# Autodesk Inventor assembly: Opentrons_Microscope_v0
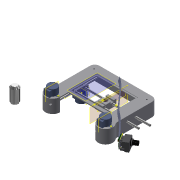
[picture p0: Inventor's stored thumbnail of the model, 180x180]
Saved by Autodesk Inventor 2019.4 (Build 234330000, 330)
## iProperties
Created: 2020-10-06
Part Number: Opentrons_Microscope_v0
Document SubType Name: Assembly
Designer: diederichbenedict
Author: diederichbenedict
## Documents named in this file (15)
- C:\Users\diederichbenedict\Dropbox\Dokumente\Promotion\PROJECTS\OPENTRONS\INVENTOR\Opentrons_Microscope_v0.iam
- C:\Users\diederichbenedict\Dropbox\Dokumente\Promotion\PROJECTS\STORMoChip\GITHUB\CAD\Nanoscopy-on-the-cheap\Workspace\00_Opticsmodule_openflexure.ipt
- C:\Users\diederichbenedict\Dropbox\Dokumente\Promotion\PROJECTS\OPENTRONS\INVENTOR\00_MTP_96-welplate.ipt
- C:\Users\diederichbenedict\Dropbox\Dokumente\Promotion\PROJECTS\OPENTRONS\INVENTOR\00_IGUS_Drylin_RJ4JP-01-06.ipt
- C:\Users\diederichbenedict\Dropbox\Dokumente\Promotion\PROJECTS\OPENTRONS\INVENTOR\00_Stepper_Motor_28BYJ-48.ipt
- C:\Users\diederichbenedict\Dropbox\Dokumente\Promotion\PROJECTS\OPENTRONS\INVENTOR\00_Thorlabs_Rod_150mm.ipt
- C:\Users\diederichbenedict\Dropbox\Dokumente\Promotion\PROJECTS\STORMoChip\GITHUB\CAD\Nanoscopy-on-the-cheap\Workspace\00_BD-DRIVE_PULLEY.ipt
- C:\Users\diederichbenedict\Dropbox\Dokumente\Promotion\PROJECTS\STORMoChip\GITHUB\CAD\Nanoscopy-on-the-cheap\Workspace\00_BD-IDLE_PULLEY.ipt
- C:\Users\diederichbenedict\Dropbox\Dokumente\Promotion\PROJECTS\OPENTRONS\INVENTOR\00_Microscope_Objective_Lens10x.ipt
- C:\Users\diederichbenedict\Dropbox\Dokumente\Promotion\PROJECTS\OPENTRONS\INVENTOR\00_Thorlabs_Rod_200mm.ipt
- C:\Users\diederichbenedict\Dropbox\Dokumente\Promotion\PROJECTS\OPENTRONS\INVENTOR\01_OTmic_BASE_v0.ipt
- C:\Users\diederichbenedict\Dropbox\Dokumente\Promotion\PROJECTS\OPENTRONS\INVENTOR\02_OTmicro_slide_y.ipt
- C:\Users\diederichbenedict\Dropbox\Dokumente\Promotion\PROJECTS\OPENTRONS\INVENTOR\03_OTmic_belt_gear.ipt
- C:\Users\diederichbenedict\Dropbox\Dokumente\Promotion\PROJECTS\OPENTRONS\INVENTOR\04_OT_mic_slide_x.ipt
- C:\Users\diederichbenedict\Dropbox\Dokumente\Promotion\PROJECTS\OPENTRONS\INVENTOR\Assembly_Opentrons_opticsmodule.iam
## Components (25 placed, 14 different names)
1. 00_Opticsmodule_openflexure:1
2. 00_MTP_96-welplate:1 — Flush:1, Flush:7, Flush:8
3. 00_Stepper_Motor_28BYJ-48:1 — Insert:2, Mate:5
4. 00_Stepper_Motor_28BYJ-48:2 — Insert:4, Mate:7
5. 00_Thorlabs_Rod_150mm:3 — Insert:1, Mate:6, Mate:9
6. 00_Thorlabs_Rod_150mm:4 — Insert:3, Mate:8, Mate:13
7. 00_BD-DRIVE_PULLEY:1 — Insert:2, Flush:3
8. 00_BD-IDLE_PULLEY:1 — Flush:3
9. 00_Microscope_Objective_Lens10x:1
10. 00_Thorlabs_Rod_200mm:3 — Insert:11, Mate:12, Mate:14
11. 01_OTmic_BASE_v0:1 — Flush:1, Insert:1, Mate:5, Insert:3, Insert:4, Mate:7, Insert:5, Angle:1, Flush:9, Flush:10
12. 00_IGUS_Drylin_RJ4JP-01-06:3 — Mate:8, Flush:4
13. 00_IGUS_Drylin_RJ4JP-01-06:4 — Mate:6, Flush:4, Flush:5
14. 00_BD-IDLE_PULLEY:2 — Insert:5
15. 00_Stepper_Motor_28BYJ-48:3 — Insert:9, Insert:10, Mate:15
16. 00_BD-DRIVE_PULLEY:2 — Mate:15, Mate:16
17. 00_Thorlabs_Rod_200mm:5 — Mate:10, Mate:11
18. 02_OTmicro_slide_y:2 — Mate:13, Mate:14, Insert:12, Angle:2
19. 02_OTmicro_slide_y:3 — Mate:9, Mate:10, Insert:9, Insert:10, Angle:1, Insert:11, Flush:5
20. 00_IGUS_Drylin_RJ4JP-01-06:5 — Mate:12, Flush:6
21. 00_IGUS_Drylin_RJ4JP-01-06:6 — Mate:11, Flush:6, Flush:7, Flush:8
22. 03_OTmic_belt_gear:1 — Insert:12, Angle:2, Insert:13
23. 00_BD-IDLE_PULLEY:3 — Insert:13, Mate:16
24. 04_OT_mic_slide_x:1 — Flush:9, Flush:10
25. Assembly_Opentrons_opticsmodule:1 [sub-assembly]
## Relationships (33: Mate 12, Insert 10, Flush 9, Angle 2)
- Flush:1: 00_MTP_96-welplate:1 ↔ 01_OTmic_BASE_v0:1
- Insert:1: 00_Thorlabs_Rod_150mm:3 ↔ 01_OTmic_BASE_v0:1
- Insert:2: 00_Stepper_Motor_28BYJ-48:1 ↔ 00_BD-DRIVE_PULLEY:1
- Mate:5 (-6 mm): 00_Stepper_Motor_28BYJ-48:1 ↔ 01_OTmic_BASE_v0:1
- Flush:3: 00_BD-DRIVE_PULLEY:1 ↔ 00_BD-IDLE_PULLEY:1
- Mate:6: 00_Thorlabs_Rod_150mm:3 ↔ 00_IGUS_Drylin_RJ4JP-01-06:4
- Insert:3: 00_Thorlabs_Rod_150mm:4 ↔ 01_OTmic_BASE_v0:1
- Insert:4: 00_Stepper_Motor_28BYJ-48:2 ↔ 01_OTmic_BASE_v0:1
- Mate:7: 00_Stepper_Motor_28BYJ-48:2 ↔ 01_OTmic_BASE_v0:1
- Insert:5: 01_OTmic_BASE_v0:1 ↔ 00_BD-IDLE_PULLEY:2
- Mate:8: 00_Thorlabs_Rod_150mm:4 ↔ 00_IGUS_Drylin_RJ4JP-01-06:3
- Flush:4: 00_IGUS_Drylin_RJ4JP-01-06:3 ↔ 00_IGUS_Drylin_RJ4JP-01-06:4
- Mate:9: 00_Thorlabs_Rod_150mm:3 ↔ 02_OTmicro_slide_y:3
- Mate:10: 00_Thorlabs_Rod_200mm:5 ↔ 02_OTmicro_slide_y:3
- Insert:9: 00_Stepper_Motor_28BYJ-48:3 ↔ 02_OTmicro_slide_y:3
- Insert:10: 00_Stepper_Motor_28BYJ-48:3 ↔ 02_OTmicro_slide_y:3
- Angle:1 (0 deg): 01_OTmic_BASE_v0:1 ↔ 02_OTmicro_slide_y:3
- Insert:11: 00_Thorlabs_Rod_200mm:3 ↔ 02_OTmicro_slide_y:3
- Flush:5 (8 mm): 00_IGUS_Drylin_RJ4JP-01-06:4 ↔ 02_OTmicro_slide_y:3
- Mate:11: 00_Thorlabs_Rod_200mm:5 ↔ 00_IGUS_Drylin_RJ4JP-01-06:6
- Mate:12: 00_Thorlabs_Rod_200mm:3 ↔ 00_IGUS_Drylin_RJ4JP-01-06:5
- Flush:6: 00_IGUS_Drylin_RJ4JP-01-06:5 ↔ 00_IGUS_Drylin_RJ4JP-01-06:6
- Mate:13: 00_Thorlabs_Rod_150mm:4 ↔ 02_OTmicro_slide_y:2
- Mate:14: 00_Thorlabs_Rod_200mm:3 ↔ 02_OTmicro_slide_y:2
- Insert:12: 02_OTmicro_slide_y:2 ↔ 03_OTmic_belt_gear:1
- Angle:2 (180 deg): 02_OTmicro_slide_y:2 ↔ 03_OTmic_belt_gear:1
- Insert:13 (-8 mm): 03_OTmic_belt_gear:1 ↔ 00_BD-IDLE_PULLEY:3
- Mate:15: 00_Stepper_Motor_28BYJ-48:3 ↔ 00_BD-DRIVE_PULLEY:2
- Mate:16: 00_BD-DRIVE_PULLEY:2 ↔ 00_BD-IDLE_PULLEY:3
- Flush:7: 00_MTP_96-welplate:1 ↔ 00_IGUS_Drylin_RJ4JP-01-06:6
- Flush:8: 00_MTP_96-welplate:1 ↔ 00_IGUS_Drylin_RJ4JP-01-06:6
- Flush:9: 01_OTmic_BASE_v0:1 ↔ 04_OT_mic_slide_x:1
- Flush:10 (-80 mm): 01_OTmic_BASE_v0:1 ↔ 04_OT_mic_slide_x:1
